# Autodesk Inventor assembly: A_openmechanism
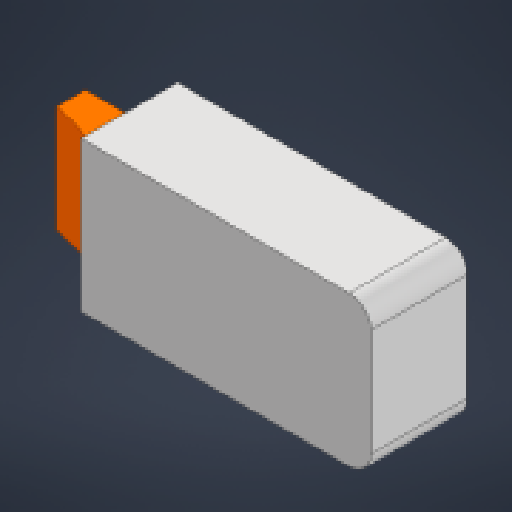
[picture p0: Inventor's stored thumbnail of the model, 512x512]
Saved by Autodesk Inventor 2026 (Build 300175000, 175)
## iProperties
Created: 2025-09-04
Part Number: A_openmechanism
Document SubType Name: Assembly
Designer: FAL
Author: FAL
## Documents named in this file (4)
- C:\Users\FAL\Projekte\Git\AEROLAB\01_AIRCRAFTS\AIR-BERT\CAD\openmechanism\A_openmechanism.iam
- C:\Users\FAL\Projekte\Git\AEROLAB\01_AIRCRAFTS\AIR-BERT\CAD\openmechanism\P_handle.ipt
- C:\Users\FAL\Projekte\Git\AEROLAB\01_AIRCRAFTS\AIR-BERT\CAD\openmechanism\P_Case.ipt
- C:\Users\FAL\Projekte\Git\AEROLAB\01_AIRCRAFTS\AIR-BERT\CAD\openmechanism\P_spring.ipt
## Components (3 placed, 3 different names)
1. P_handle:1 — Passend:1, Fluchtend:7
2. P_Case:1 — Fluchtend:1, Fluchtend:2, Fluchtend:3, Fluchtend:5, Passend:1
3. P_spring:1 — Fluchtend:5, Fluchtend:6
## Relationships (7: Flush 6, Mate 1)
- Fluchtend:1 [Flush]: P_Case:1
- Fluchtend:2 [Flush]: P_Case:1
- Fluchtend:3 [Flush]: P_Case:1
- Fluchtend:5 [Flush]: P_Case:1 ↔ P_spring:1
- Fluchtend:6 [Flush]: P_spring:1
- Passend:1 [Mate]: P_handle:1 ↔ P_Case:1
- Fluchtend:7 [Flush]: P_handle:1
